# Autodesk Inventor assembly: Cabinet
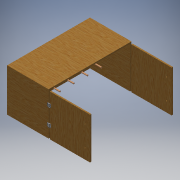
[picture p0: Inventor's stored thumbnail of the model, 180x180]
Saved by Autodesk Inventor 2019 (Build 230136000, 136)
## iProperties
Created: 2018-09-21
Part Number: Cabinet
Document SubType Name: Assembly
Designer: user
Author: user
## Documents named in this file (7)
- C:\Users\user\Desktop\Roombotics\Cabinet.iam
- C:\Users\user\Desktop\College\IPRO\SwerveProto\Wall1.ipt
- C:\Users\user\Desktop\College\IPRO\SwerveProto\Wall2.ipt
- C:\Users\user\Desktop\College\IPRO\SwerveProto\Door1.ipt
- C:\Users\user\Downloads\2190A120_FRICTION HINGE.ipt
- C:\Users\user\Desktop\College\IPRO\SwerveProto\Top.ipt
- C:\Users\user\Desktop\College\IPRO\SwerveProto\Dowel.ipt
## Components (11 placed, 6 different names)
1. Wall1:1 — Flush:1, Mate:5, Flush:7, Flush:8, Mate:6, Flush:9, Flush:10, Mate:7, Flush:11
2. Wall2:1 — Flush:1, Rigid:1, Flush:12, Flush:13
3. Wall1:2 — Rigid:1, Mate:1, Flush:2, Flush:3, Mate:2, Flush:4, Flush:5, Mate:3, Flush:6
4. 2190A120_FRICTION HINGE:1 — Mate:1, Flush:2, Flush:3
5. 2190A120_FRICTION HINGE:2 — Mate:2, Flush:4, Flush:5, Mate:4
6. 2190A120_FRICTION HINGE:3 — Mate:6, Flush:9, Flush:10
7. 2190A120_FRICTION HINGE:4 — Mate:5, Flush:7, Flush:8, Mate:8
8. Door1:2 — Mate:3, Mate:4, Flush:6
9. Door1:3 — Mate:7, Flush:11, Mate:8
10. Top:1 — Flush:12
11. Dowel:1 — Flush:13
## Relationships (22: Flush 13, Mate 8, WeldJoint 1)
- Flush:1: Wall1:1 ↔ Wall2:1
- Rigid:1 [WeldJoint]: Wall2:1 ↔ Wall1:2
- Mate:1: Wall1:2 ↔ 2190A120_FRICTION HINGE:1
- Flush:2 (152.4 mm): Wall1:2 ↔ 2190A120_FRICTION HINGE:1
- Flush:3: Wall1:2 ↔ 2190A120_FRICTION HINGE:1
- Mate:2: Wall1:2 ↔ 2190A120_FRICTION HINGE:2
- Flush:4 (152.4 mm): Wall1:2 ↔ 2190A120_FRICTION HINGE:2
- Flush:5: Wall1:2 ↔ 2190A120_FRICTION HINGE:2
- Mate:3 (19.05 mm): Wall1:2 ↔ Door1:2
- Mate:4: 2190A120_FRICTION HINGE:2 ↔ Door1:2
- Flush:6: Wall1:2 ↔ Door1:2
- Mate:5: Wall1:1 ↔ 2190A120_FRICTION HINGE:4
- Flush:7 (152.4 mm): Wall1:1 ↔ 2190A120_FRICTION HINGE:4
- Flush:8: Wall1:1 ↔ 2190A120_FRICTION HINGE:4
- Mate:6: Wall1:1 ↔ 2190A120_FRICTION HINGE:3
- Flush:9 (152.4 mm): Wall1:1 ↔ 2190A120_FRICTION HINGE:3
- Flush:10: Wall1:1 ↔ 2190A120_FRICTION HINGE:3
- Mate:7 (19.05 mm): Wall1:1 ↔ Door1:3
- Flush:11: Wall1:1 ↔ Door1:3
- Mate:8: 2190A120_FRICTION HINGE:4 ↔ Door1:3
- Flush:12: Wall2:1 ↔ Top:1
- Flush:13: Wall2:1 ↔ Dowel:1
